# Autodesk Inventor assembly: topassy
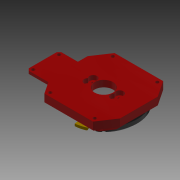
[picture p0: Inventor's stored thumbnail of the model, 180x180]
Saved by Autodesk Inventor 2018 (Build 220112000, 112)
## iProperties
Created: 2019-02-21
Part Number: topassy
Material: 一般
Document SubType Name: Assembly
Designer: ku_sk
Author: ku_sk
## Documents named in this file (5)
- E:\windows\Documents\Inventor\Content Center Files\bay shooter\parts\toptest.iam
- E:\windows\Documents\Inventor\Content Center Files\bay shooter\parts\topcover.ipt
- E:\windows\Documents\Inventor\Content Center Files\bay shooter\parts\skyrimlogo2_1_9.ipt
- E:\windows\Documents\Inventor\Content Center Files\bay shooter\parts\ring.ipt
- E:\windows\Documents\Inventor\Content Center Files\bay shooter\parts\cover.ipt
## Components (4 placed, 4 different names)
1. topcover:1 — メイト:1, 角度:1, メイト:2, メイト:3, メイト:4, メイト:5, メイト:6, メイト:7, メイト:10, メイト:11, メイト:12
2. skyrimlogo2_1_9:1 — メイト:1, 角度:1, メイト:2
3. ring:1 — メイト:6, メイト:7
4. cover:1 — メイト:10, メイト:11, メイト:12
## Relationships (11: Mate 10, Angle 1)
- メイト:1 [Mate] (-1.2 mm): topcover:1 ↔ skyrimlogo2_1_9:1
- 角度:1 [Angle] (26.37 deg): topcover:1 ↔ skyrimlogo2_1_9:1
- メイト:2 [Mate]: topcover:1 ↔ skyrimlogo2_1_9:1
- メイト:3 [Mate]: topcover:1
- メイト:4 [Mate]: topcover:1
- メイト:5 [Mate]: topcover:1
- メイト:6 [Mate]: topcover:1 ↔ ring:1
- メイト:7 [Mate]: topcover:1 ↔ ring:1
- メイト:10 [Mate]: topcover:1 ↔ cover:1
- メイト:11 [Mate]: topcover:1 ↔ cover:1
- メイト:12 [Mate]: topcover:1 ↔ cover:1
